# Autodesk Inventor assembly: CaseA
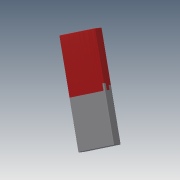
[picture p0: Inventor's stored thumbnail of the model, 180x180]
Saved by Autodesk Inventor 2019 (Build 230136000, 136)
## iProperties
Created: 2019-05-06
Part Number: CaseA
Document SubType Name: Assembly
Designer: giacomo
Author: giacomo
## Documents named in this file (3)
- D:\Hobby\Inventor\Case 3Dprinted\A\CaseA.iam
- D:\Hobby\Inventor\Case 3Dprinted\A\Case_A1.ipt
- D:\Hobby\Inventor\Case 3Dprinted\A\Case_A2.ipt
## Components (2 placed, 2 different names)
1. Case_A1:1 — Flush:1, Mate:1, Flush:2
2. Case_A2:1 — Flush:1, Mate:1, Flush:2
## Relationships (3: Flush 2, Mate 1)
- Flush:1: Case_A1:1 ↔ Case_A2:1
- Mate:1: Case_A1:1 ↔ Case_A2:1
- Flush:2: Case_A1:1 ↔ Case_A2:1
